# Autodesk Inventor assembly: ShoulderLeft
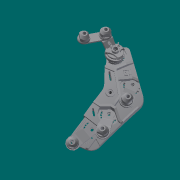
[picture p0: Inventor's stored thumbnail of the model, 180x180]
Saved by Autodesk Inventor 2015 SP1 (Build 190203100, 203)
## iProperties
Created: 2016-10-02
Part Number: ShoulderLeft
Document SubType Name: Assembly
Designer: Val
Author: Val
## Documents named in this file (8)
- C:\Users\Val\Desktop\ExoGit\elysium-max-exoskeleton\src\Assemblies\ShoulderLeft.iam
- C:\Users\Val\Desktop\ExoGit\elysium-max-exoskeleton\src\ShoulderLeft.ipt
- C:\Users\Val\Desktop\ExoGit\elysium-max-exoskeleton\src\ShoulderCogLarge.ipt
- C:\Users\Val\Desktop\ExoGit\elysium-max-exoskeleton\src\ShoulderCogSmall.ipt
- C:\Users\Val\Desktop\ExoGit\elysium-max-exoskeleton\src\BackConnector.ipt
- C:\Users\Val\Desktop\ExoGit\elysium-max-exoskeleton\src\BackSideConnector.ipt
- C:\Users\Val\Desktop\ExoGit\elysium-max-exoskeleton\src\Assemblies\ShoulderConnector.iam
- C:\Users\Val\Desktop\ExoGit\elysium-max-exoskeleton\src\SpacerShort.ipt
## Components (15 placed, 7 different names)
1. ShoulderLeft:1 — Mate:1, Mate:2, Mate:3, Mate:4, Mate:5, Mate:6, Mate:7, Mate:8, Mate:9, Mate:10, Mate:13, Mate:15, Mate:17
2. ShoulderCogLarge:1 — Mate:1, Mate:2
3. ShoulderCogSmall:1 — Mate:7, Mate:8, Mate:14
4. ShoulderCogSmall:2 — Mate:5, Mate:6, Mate:16
5. ShoulderCogSmall:3 — Mate:3, Mate:4, Mate:18
6. BackConnector:1 — Mate:13, Mate:14, Mate:23, Mate:26
7. BackSideConnector:1 — Mate:11, Mate:12, Mate:19, Mate:20, Mate:21, Mate:22
8. BackConnector:2 — Mate:15, Mate:16, Mate:25, Mate:27
9. BackConnector:3 — Mate:17, Mate:18, Mate:24, Mate:28
10. ShoulderConnectorSplit:1 [sub-assembly] — Mate:9, Mate:10, Mate:11, Mate:12
11. SpacerShort:1 — Mate:19, Mate:21
12. SpacerShort:2 — Mate:20, Mate:22
13. SpacerShort:3 — Mate:23, Mate:26
14. SpacerShort:4 — Mate:25, Mate:27
15. SpacerShort:5 — Mate:24, Mate:28
## Relationships (28: Mate 28)
- Mate:1: ShoulderLeft:1 ↔ ShoulderCogLarge:1
- Mate:2: ShoulderLeft:1 ↔ ShoulderCogLarge:1
- Mate:3: ShoulderLeft:1 ↔ ShoulderCogSmall:3
- Mate:4: ShoulderLeft:1 ↔ ShoulderCogSmall:3
- Mate:5: ShoulderLeft:1 ↔ ShoulderCogSmall:2
- Mate:6: ShoulderLeft:1 ↔ ShoulderCogSmall:2
- Mate:7: ShoulderLeft:1 ↔ ShoulderCogSmall:1
- Mate:8: ShoulderLeft:1 ↔ ShoulderCogSmall:1
- Mate:9: ShoulderLeft:1 ↔ ShoulderConnectorSplit:1
- Mate:10: ShoulderLeft:1 ↔ ShoulderConnectorSplit:1
- Mate:11: BackSideConnector:1 ↔ ShoulderConnectorSplit:1
- Mate:12: BackSideConnector:1 ↔ ShoulderConnectorSplit:1
- Mate:13: ShoulderLeft:1 ↔ BackConnector:1
- Mate:14: ShoulderCogSmall:1 ↔ BackConnector:1
- Mate:15: ShoulderLeft:1 ↔ BackConnector:2
- Mate:16: ShoulderCogSmall:2 ↔ BackConnector:2
- Mate:17: ShoulderLeft:1 ↔ BackConnector:3
- Mate:18: ShoulderCogSmall:3 ↔ BackConnector:3
- Mate:19: BackSideConnector:1 ↔ SpacerShort:1
- Mate:20: BackSideConnector:1 ↔ SpacerShort:2
- Mate:21: BackSideConnector:1 ↔ SpacerShort:1
- Mate:22: BackSideConnector:1 ↔ SpacerShort:2
- Mate:23: BackConnector:1 ↔ SpacerShort:3
- Mate:24: BackConnector:3 ↔ SpacerShort:5
- Mate:25: BackConnector:2 ↔ SpacerShort:4
- Mate:26: BackConnector:1 ↔ SpacerShort:3
- Mate:27: BackConnector:2 ↔ SpacerShort:4
- Mate:28: BackConnector:3 ↔ SpacerShort:5
